# Autodesk Inventor assembly: iPadHolderAssembly
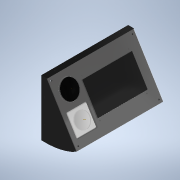
[picture p0: Inventor's stored thumbnail of the model, 180x180]
Saved by Autodesk Inventor 2021 (Build 250183000, 183)
## iProperties
Created: 2020-11-06
Part Number: iPadHolderAssembly
Document SubType Name: Assembly
Designer: gisen
Author: gisen
## Documents named in this file (6)
- D:\GitProjects\CAD-Data\CuboidAccessories\SecurityBox\Assemblies\DisplayHolderAssembly.iam
- D:\GitProjects\CAD-Data\CuboidAccessories\SecurityBox\3DPrintedParts\DisplayHolder.ipt
- D:\GitProjects\CAD-Data\Devices\Microphone\Microphone_iGOKU.ipt
- D:\GitProjects\CAD-Data\Devices\Display\Display_EVICIV7Inch.ipt
- D:\GitProjects\CAD-Data\Devices\Button\Button.ipt
- D:\GitProjects\CAD-Data\CuboidAccessories\SecurityBox\Plates\DisplayHolderCoverPlate.ipt
## Components (5 placed, 5 different names)
1. DisplayHolder:1 — メイト:4, メイト:7, フラッシュ:1, フラッシュ:3, メイト:8, メイト:9, フラッシュ:5, メイト:11, メイト:13, メイト:14, メイト:15, メイト:16, メイト:17, フラッシュ:6, メイト:18
2. Microphone_iGOKU:1 — メイト:7, メイト:9, メイト:15
3. Display_EVICIV7Inch:1 — フラッシュ:1, メイト:8, フラッシュ:5
4. Button:1 — フラッシュ:3, メイト:11, メイト:16
5. DisplayHolderCoverPlate:1 — メイト:17, フラッシュ:6, メイト:18
## Relationships (15: Mate 11, Flush 4)
- メイト:4 [Mate]: DisplayHolder:1
- メイト:7 [Mate] (-5.5 mm): DisplayHolder:1 ↔ Microphone_iGOKU:1
- フラッシュ:1 [Flush] (2 mm): DisplayHolder:1 ↔ Display_EVICIV7Inch:1
- フラッシュ:3 [Flush] (1 mm): DisplayHolder:1 ↔ Button:1
- メイト:8 [Mate]: DisplayHolder:1 ↔ Display_EVICIV7Inch:1
- メイト:9 [Mate] (-50 mm): DisplayHolder:1 ↔ Microphone_iGOKU:1
- フラッシュ:5 [Flush] (30 mm): DisplayHolder:1 ↔ Display_EVICIV7Inch:1
- メイト:11 [Mate] (-50 mm): DisplayHolder:1 ↔ Button:1
- メイト:13 [Mate]: DisplayHolder:1
- メイト:14 [Mate]: DisplayHolder:1
- メイト:15 [Mate]: DisplayHolder:1 ↔ Microphone_iGOKU:1
- メイト:16 [Mate] (-60 mm): DisplayHolder:1 ↔ Button:1
- メイト:17 [Mate]: DisplayHolder:1 ↔ DisplayHolderCoverPlate:1
- フラッシュ:6 [Flush]: DisplayHolder:1 ↔ DisplayHolderCoverPlate:1
- メイト:18 [Mate]: DisplayHolder:1 ↔ DisplayHolderCoverPlate:1
